# Autodesk Inventor assembly: Completed Locked CubeSat Assembly
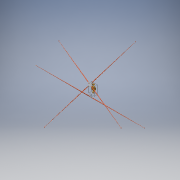
[picture p0: Inventor's stored thumbnail of the model, 180x180]
Saved by Autodesk Inventor 2016 (Build 200138000, 138)
## iProperties
Created: 2015-12-30
Part Number: Completed Locked CubeSat Assembly
Document SubType Name: Assembly
Designer: jonathan
Author: jonathan
## Documents named in this file (5)
- C:\Users\jonathan\Dropbox\Satellite\CAD\Completed Locked CubeSat Assembly.iam
- C:\Users\jonathan\Dropbox\Satellite\CAD\Locked CubeSat Assembly Frame.iam
- C:\Users\jonathan\Dropbox\Satellite\CAD\Large Flywheel.ipt
- C:\Users\jonathan\Dropbox\Satellite\CAD\Small Flywheel.ipt
- C:\Users\jonathan\Dropbox\Satellite\CAD\Spinning Platform.iam
## Components (6 placed, 4 different names)
1. Locked CubeSat Assembly Frame:1 [sub-assembly] — Mate:3, Mate:4, Mate:5, Mate:6, Mate:7, Mate:8, Mate:9, Mate:10, Mate:11, Mate:12
2. Large Flywheel:1 — Mate:3, Mate:4
3. Small Flywheel:1 — Mate:5, Mate:6
4. Small Flywheel:2 — Mate:7, Mate:8
5. Spinning Platform:3 [sub-assembly] — Mate:9, Mate:10
6. Spinning Platform:4 [sub-assembly] — Mate:11, Mate:12
## Relationships (10: Mate 10)
- Mate:3: Locked CubeSat Assembly Frame:1 ↔ Large Flywheel:1
- Mate:4: Locked CubeSat Assembly Frame:1 ↔ Large Flywheel:1
- Mate:5: Locked CubeSat Assembly Frame:1 ↔ Small Flywheel:1
- Mate:6: Locked CubeSat Assembly Frame:1 ↔ Small Flywheel:1
- Mate:7: Locked CubeSat Assembly Frame:1 ↔ Small Flywheel:2
- Mate:8: Locked CubeSat Assembly Frame:1 ↔ Small Flywheel:2
- Mate:9: Locked CubeSat Assembly Frame:1 ↔ Spinning Platform:3
- Mate:10: Locked CubeSat Assembly Frame:1 ↔ Spinning Platform:3
- Mate:11: Locked CubeSat Assembly Frame:1 ↔ Spinning Platform:4
- Mate:12: Locked CubeSat Assembly Frame:1 ↔ Spinning Platform:4
